# Autodesk Inventor assembly: main track assembly
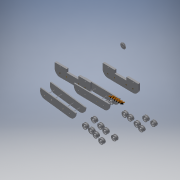
[picture p0: Inventor's stored thumbnail of the model, 180x180]
Saved by Autodesk Inventor 2019 (Build 230136000, 136)
## iProperties
Created: 2019-04-25
Part Number: main track assembly
Document SubType Name: Assembly
Designer: User
Author: User
## Documents named in this file (9)
- C:\Robotics\CAD\2019-20_CAD\offseason\random ideas\mecanum tracks\main track assembly.iam
- D:\The THING\right assembly.iam
- C:\Robotics\CAD\2019-20_CAD\offseason\random ideas\side drivetrain piece (8 wheel macanum).ipt
- C:\Robotics\CAD\2019-20_CAD\offseason\random ideas\side drivetrain piece (8 wheel macanum) - Copy.ipt
- C:\Robotics\CAD\COTSParts\Tetrix\Tetrix tread sprocket.ipt
- C:\Robotics\CAD\COTSParts\Tetrix\Bronze bushing.ipt
- C:\Robotics\CAD\COTSParts\Tetrix\Tetrix shaft 250mm.ipt
- C:\Robotics\CAD\COTSParts\Tetrix\Tetrix shaft collar.ipt
- C:\Robotics\CAD\2019-20_CAD\offseason\random ideas\mecanum tracks\tread roller assembly.iam
## Components (80 placed, 8 different names)
1. right assembly:1 [sub-assembly]
2. side drivetrain piece (8 wheel macanum):1 — Insert:9, Insert:10, Insert:11, Insert:12, Insert:29, Insert:30, Insert:31, Insert:32
3. side drivetrain piece (8 wheel macanum):2 — Insert:1, Insert:2, Insert:3, Insert:4, Insert:21, Insert:22, Insert:23, Insert:24
4. side drivetrain piece (8 wheel macanum) - Copy:1 — Insert:5, Insert:6, Insert:7, Insert:8
5. side drivetrain piece (8 wheel macanum) - Copy:2 — Insert:17, Insert:18, Insert:19, Insert:20
6. side drivetrain piece (8 wheel macanum) - Copy:3 — Insert:25, Insert:26, Insert:27, Insert:28, Mate:31
7. side drivetrain piece (8 wheel macanum) - Copy:4 — Insert:13, Insert:14, Insert:15, Insert:16, Mate:29
8. Tetrix tread sprocket:3
9. Bronze bushing:1 — Insert:12
10. Bronze bushing:2 — Insert:11
11. Bronze bushing:3 — Insert:10
12. Bronze bushing:4 — Insert:8, Mate:16, Mate:17
13. Bronze bushing:5 — Insert:7, Mate:22
14. Bronze bushing:6 — Insert:6, Mate:25
15. Bronze bushing:7 — Insert:5, Mate:20
16. Bronze bushing:8 — Insert:4
17. Bronze bushing:9 — Insert:3
18. Bronze bushing:10 — Insert:2
19. Bronze bushing:11 — Insert:1
20. Bronze bushing:12 — Insert:15, Mate:11, Mate:13
21. Bronze bushing:13 — Insert:16, Mate:1, Mate:2
22. Bronze bushing:14 — Insert:14, Mate:8, Mate:10
23. Bronze bushing:15 — Insert:13, Mate:5, Mate:6
24. Bronze bushing:16 — Insert:9
25. Bronze bushing:17 — Insert:17, Mate:14, Mate:15, Mate:18
26. Bronze bushing:18 — Insert:20, Mate:19
27. Bronze bushing:19 — Insert:23
28. Bronze bushing:20 — Insert:24
29. Bronze bushing:21 — Insert:18, Mate:21, Mate:23
30. Bronze bushing:22 — Insert:19, Mate:24, Mate:26
31. Bronze bushing:23 — Insert:21
32. Bronze bushing:24 — Insert:22
33. Bronze bushing:25 — Insert:25, Mate:3, Mate:4
34. Bronze bushing:26 — Insert:26, Mate:12
35. Bronze bushing:27 — Insert:27, Mate:9
36. Bronze bushing:28 — Insert:28, Mate:7
37. Bronze bushing:29 — Insert:29, Mate:28
38. Bronze bushing:30 — Insert:31
39. Bronze bushing:31 — Insert:30
40. Bronze bushing:32 — Insert:32, Mate:27
41. Tetrix shaft 250mm:1 — Insert:33, Insert:41, Mate:5, Mate:7, Mate:28, Mate:30, Mate:32
42. Tetrix shaft 250mm:2 — Insert:34, Insert:42, Mate:8, Mate:9
43. Tetrix shaft 250mm:3 — Insert:35, Insert:43, Mate:11, Mate:12
44. Tetrix shaft 250mm:4 — Insert:36, Insert:44, Mate:15, Mate:16
45. Tetrix shaft 250mm:5 — Insert:37, Insert:45, Mate:1, Mate:3, Mate:27
46. Tetrix shaft 250mm:6 — Insert:38, Insert:46, Mate:24, Mate:25
47. Tetrix shaft 250mm:7 — Insert:39, Insert:47, Mate:21, Mate:22
48. Tetrix shaft 250mm:8 — Insert:40, Insert:48, Mate:19, Mate:20
49. Tetrix shaft collar:1 — Insert:37, Mate:4
50. Tetrix shaft collar:2 — Insert:38
51. Tetrix shaft collar:3 — Insert:39
52. Tetrix shaft collar:4 — Insert:40, Mate:14
53. Tetrix shaft collar:5 — Insert:45, Mate:2
54. Tetrix shaft collar:6 — Insert:46, Mate:26
55. Tetrix shaft collar:7 — Insert:47, Mate:23
56. Tetrix shaft collar:8 — Insert:48
57. Tetrix shaft collar:9 — Insert:33
58. Tetrix shaft collar:10 — Insert:34, Mate:10
59. Tetrix shaft collar:11 — Insert:35
60. Tetrix shaft collar:12 — Insert:36, Mate:17
61. Tetrix shaft collar:13 — Insert:41, Mate:6
62. Tetrix shaft collar:14 — Insert:42
63. Tetrix shaft collar:15 — Insert:43, Mate:13
64. Tetrix shaft collar:16 — Insert:44, Mate:18
65. tread roller assembly:1 [sub-assembly] — Mate:29, Mate:30
66. tread roller assembly:2 [sub-assembly] — Mate:31, Mate:32
67. tread roller assembly:3 [sub-assembly]
68. tread roller assembly:4 [sub-assembly]
69. tread roller assembly:5 [sub-assembly]
70. tread roller assembly:6 [sub-assembly]
71. tread roller assembly:7 [sub-assembly]
72. tread roller assembly:8 [sub-assembly]
73. tread roller assembly:9 [sub-assembly]
74. tread roller assembly:10 [sub-assembly]
75. tread roller assembly:11 [sub-assembly]
76. tread roller assembly:12 [sub-assembly]
77. tread roller assembly:13 [sub-assembly]
78. tread roller assembly:14 [sub-assembly]
79. tread roller assembly:15 [sub-assembly]
80. tread roller assembly:16 [sub-assembly]
## Relationships (80: Insert 48, Mate 32)
- Insert:1: side drivetrain piece (8 wheel macanum):2 ↔ Bronze bushing:11
- Insert:2: side drivetrain piece (8 wheel macanum):2 ↔ Bronze bushing:10
- Insert:3: side drivetrain piece (8 wheel macanum):2 ↔ Bronze bushing:9
- Insert:4: side drivetrain piece (8 wheel macanum):2 ↔ Bronze bushing:8
- Insert:5: side drivetrain piece (8 wheel macanum) - Copy:1 ↔ Bronze bushing:7
- Insert:6: side drivetrain piece (8 wheel macanum) - Copy:1 ↔ Bronze bushing:6
- Insert:7: side drivetrain piece (8 wheel macanum) - Copy:1 ↔ Bronze bushing:5
- Insert:8: side drivetrain piece (8 wheel macanum) - Copy:1 ↔ Bronze bushing:4
- Insert:9: side drivetrain piece (8 wheel macanum):1 ↔ Bronze bushing:16
- Insert:10: side drivetrain piece (8 wheel macanum):1 ↔ Bronze bushing:3
- Insert:11: side drivetrain piece (8 wheel macanum):1 ↔ Bronze bushing:2
- Insert:12: side drivetrain piece (8 wheel macanum):1 ↔ Bronze bushing:1
- Insert:13: side drivetrain piece (8 wheel macanum) - Copy:4 ↔ Bronze bushing:15
- Insert:14: side drivetrain piece (8 wheel macanum) - Copy:4 ↔ Bronze bushing:14
- Insert:15: side drivetrain piece (8 wheel macanum) - Copy:4 ↔ Bronze bushing:12
- Insert:16: side drivetrain piece (8 wheel macanum) - Copy:4 ↔ Bronze bushing:13
- Insert:17: side drivetrain piece (8 wheel macanum) - Copy:2 ↔ Bronze bushing:17
- Insert:18: side drivetrain piece (8 wheel macanum) - Copy:2 ↔ Bronze bushing:21
- Insert:19: side drivetrain piece (8 wheel macanum) - Copy:2 ↔ Bronze bushing:22
- Insert:20: side drivetrain piece (8 wheel macanum) - Copy:2 ↔ Bronze bushing:18
- Insert:21: side drivetrain piece (8 wheel macanum):2 ↔ Bronze bushing:23
- Insert:22: side drivetrain piece (8 wheel macanum):2 ↔ Bronze bushing:24
- Insert:23: side drivetrain piece (8 wheel macanum):2 ↔ Bronze bushing:19
- Insert:24: side drivetrain piece (8 wheel macanum):2 ↔ Bronze bushing:20
- Insert:25: side drivetrain piece (8 wheel macanum) - Copy:3 ↔ Bronze bushing:25
- Insert:26: side drivetrain piece (8 wheel macanum) - Copy:3 ↔ Bronze bushing:26
- Insert:27: side drivetrain piece (8 wheel macanum) - Copy:3 ↔ Bronze bushing:27
- Insert:28: side drivetrain piece (8 wheel macanum) - Copy:3 ↔ Bronze bushing:28
- Insert:29: side drivetrain piece (8 wheel macanum):1 ↔ Bronze bushing:29
- Insert:30: side drivetrain piece (8 wheel macanum):1 ↔ Bronze bushing:31
- Insert:31: side drivetrain piece (8 wheel macanum):1 ↔ Bronze bushing:30
- Insert:32: side drivetrain piece (8 wheel macanum):1 ↔ Bronze bushing:32
- Insert:33: Tetrix shaft 250mm:1 ↔ Tetrix shaft collar:9
- Insert:34: Tetrix shaft 250mm:2 ↔ Tetrix shaft collar:10
- Insert:35: Tetrix shaft 250mm:3 ↔ Tetrix shaft collar:11
- Insert:36: Tetrix shaft 250mm:4 ↔ Tetrix shaft collar:12
- Insert:37: Tetrix shaft 250mm:5 ↔ Tetrix shaft collar:1
- Insert:38: Tetrix shaft 250mm:6 ↔ Tetrix shaft collar:2
- Insert:39: Tetrix shaft 250mm:7 ↔ Tetrix shaft collar:3
- Insert:40: Tetrix shaft 250mm:8 ↔ Tetrix shaft collar:4
- Insert:41: Tetrix shaft 250mm:1 ↔ Tetrix shaft collar:13
- Insert:42: Tetrix shaft 250mm:2 ↔ Tetrix shaft collar:14
- Insert:43: Tetrix shaft 250mm:3 ↔ Tetrix shaft collar:15
- Insert:44: Tetrix shaft 250mm:4 ↔ Tetrix shaft collar:16
- Insert:45: Tetrix shaft 250mm:5 ↔ Tetrix shaft collar:5
- Insert:46: Tetrix shaft 250mm:6 ↔ Tetrix shaft collar:6
- Insert:47: Tetrix shaft 250mm:7 ↔ Tetrix shaft collar:7
- Insert:48: Tetrix shaft 250mm:8 ↔ Tetrix shaft collar:8
- Mate:1: Bronze bushing:13 ↔ Tetrix shaft 250mm:5
- Mate:2: Bronze bushing:13 ↔ Tetrix shaft collar:5
- Mate:3: Bronze bushing:25 ↔ Tetrix shaft 250mm:5
- Mate:4: Bronze bushing:25 ↔ Tetrix shaft collar:1
- Mate:5: Bronze bushing:15 ↔ Tetrix shaft 250mm:1
- Mate:6: Bronze bushing:15 ↔ Tetrix shaft collar:13
- Mate:7: Bronze bushing:28 ↔ Tetrix shaft 250mm:1
- Mate:8: Bronze bushing:14 ↔ Tetrix shaft 250mm:2
- Mate:9: Bronze bushing:27 ↔ Tetrix shaft 250mm:2
- Mate:10: Bronze bushing:14 ↔ Tetrix shaft collar:10
- Mate:11: Bronze bushing:12 ↔ Tetrix shaft 250mm:3
- Mate:12: Bronze bushing:26 ↔ Tetrix shaft 250mm:3
- Mate:13: Bronze bushing:12 ↔ Tetrix shaft collar:15
- Mate:14: Bronze bushing:17 ↔ Tetrix shaft collar:4
- Mate:15: Bronze bushing:17 ↔ Tetrix shaft 250mm:4
- Mate:16: Bronze bushing:4 ↔ Tetrix shaft 250mm:4
- Mate:17: Bronze bushing:4 ↔ Tetrix shaft collar:12
- Mate:18: Bronze bushing:17 ↔ Tetrix shaft collar:16
- Mate:19: Bronze bushing:18 ↔ Tetrix shaft 250mm:8
- Mate:20: Bronze bushing:7 ↔ Tetrix shaft 250mm:8
- Mate:21: Bronze bushing:21 ↔ Tetrix shaft 250mm:7
- Mate:22: Bronze bushing:5 ↔ Tetrix shaft 250mm:7
- Mate:23: Bronze bushing:21 ↔ Tetrix shaft collar:7
- Mate:24: Bronze bushing:22 ↔ Tetrix shaft 250mm:6
- Mate:25: Bronze bushing:6 ↔ Tetrix shaft 250mm:6
- Mate:26: Bronze bushing:22 ↔ Tetrix shaft collar:6
- Mate:27: Bronze bushing:32 ↔ Tetrix shaft 250mm:5
- Mate:28: Bronze bushing:29 ↔ Tetrix shaft 250mm:1
- Mate:29: side drivetrain piece (8 wheel macanum) - Copy:4 ↔ tread roller assembly:1
- Mate:30: Tetrix shaft 250mm:1 ↔ tread roller assembly:1
- Mate:31: side drivetrain piece (8 wheel macanum) - Copy:3 ↔ tread roller assembly:2
- Mate:32: Tetrix shaft 250mm:1 ↔ tread roller assembly:2
